# Autodesk Inventor assembly: sec_floor
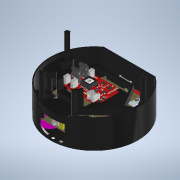
[picture p0: Inventor's stored thumbnail of the model, 180x180]
Saved by Autodesk Inventor 2020.4 (Build 244396000, 396)
## iProperties
Created: 2021-11-24
Part Number: sec_floor
Document SubType Name: Assembly
Designer: Acer
Author: Acer
## Documents named in this file (11)
- C:\Users\Acer\Documents\MATLAB\Doutorado\CAD\Inventor\sec_floor\sec_floor.iam
- C:\Users\Acer\Documents\MATLAB\Doutorado\CAD\Inventor\sec_floor\plate_sec_floor.ipt
- C:\Users\Acer\Documents\MATLAB\Doutorado\CAD\Inventor\sec_floor\SupportFirstToSecond.ipt
- C:\Users\Acer\Documents\MATLAB\Doutorado\CAD\Inventor\sec_floor\SupportSecondToCoverNew.ipt
- C:\Users\Acer\Documents\MATLAB\Doutorado\CAD\Inventor\sec_floor\MainboardSpacer.ipt
- C:\Users\Acer\Documents\MATLAB\Doutorado\CAD\Inventor\sec_floor\KickerBoard\KickerBoard_V1.1.iam
- C:\Users\Acer\Documents\MATLAB\Doutorado\CAD\Inventor\sec_floor\MainBoard\MainBoard_V1.1.iam
- C:\Users\Acer\Documents\MATLAB\Doutorado\CAD\Inventor\sec_floor\CoverNew.ipt
- C:\Users\Acer\Documents\MATLAB\Doutorado\CAD\Inventor\sec_floor\tag_green.ipt
- C:\Users\Acer\Documents\MATLAB\Doutorado\CAD\Inventor\sec_floor\tag_magenta.ipt
- C:\Users\Acer\Documents\MATLAB\Doutorado\CAD\Inventor\sec_floor\tag_yellow.ipt
## Components (19 placed, 10 different names)
1. plate_sec_floor:1 — Mate:1, Mate:2, Mate:3, Mate:4, Angle:1, Angle:2, Angle:3, Angle:4, Mate:5, Mate:6, Mate:7, Mate:8, Mate:9, Mate:10, Angle:5, Angle:6, Mate:11, Mate:12, Mate:13, Mate:14, Mate:15, Mate:16, Angle:7, Angle:8, Angle:9, Angle:10, Mate:17, Mate:18, Mate:19, Mate:20, Mate:21, Mate:22, Mate:23, Angle:11
2. SupportFirstToSecond:1 — Mate:1, Angle:4, Mate:5
3. SupportFirstToSecond:2 — Mate:2, Angle:3, Mate:8
4. SupportFirstToSecond:3 — Mate:4, Angle:1, Mate:6
5. SupportFirstToSecond:4 — Mate:3, Angle:2, Mate:7
6. SupportSecondToCoverNew:1 — Mate:9, Angle:5, Mate:12, Mate:28
7. SupportSecondToCoverNew:2 — Mate:10, Angle:6, Mate:11, Mate:27
8. MainboardSpacer:1 — Mate:13, Angle:7, Mate:19
9. MainboardSpacer:2 — Mate:14, Angle:8, Mate:17, Mate:26
10. MainboardSpacer:3 — Mate:16, Angle:9, Mate:20, Mate:24
11. MainboardSpacer:4 — Mate:15, Angle:10, Mate:18, Mate:25
12. KickerBoard_V1.1:1 [sub-assembly] — Mate:21, Mate:22, Mate:23
13. MainBoard_V1.1:1 [sub-assembly] — Mate:24, Mate:25, Mate:26
14. CoverNew:1 — Mate:27, Angle:11, Mate:28, Mate:29, Mate:30, Mate:31, Mate:32, Mate:33, Mate:34, Mate:35, Mate:36, Mate:37, Mate:38
15. tag_green:1 — Mate:31, Mate:36
16. tag_green:2 — Mate:32, Mate:35
17. tag_magenta:1 — Mate:33, Mate:37
18. tag_magenta:2 — Mate:34, Mate:38
19. tag_yellow:1 — Mate:29, Mate:30
## Relationships (49: Mate 38, Angle 11)
- Mate:1: plate_sec_floor:1 ↔ SupportFirstToSecond:1
- Mate:2: plate_sec_floor:1 ↔ SupportFirstToSecond:2
- Mate:3: plate_sec_floor:1 ↔ SupportFirstToSecond:4
- Mate:4: plate_sec_floor:1 ↔ SupportFirstToSecond:3
- Angle:1 (0 deg): plate_sec_floor:1 ↔ SupportFirstToSecond:3
- Angle:2 (0 deg): plate_sec_floor:1 ↔ SupportFirstToSecond:4
- Angle:3 (0 deg): plate_sec_floor:1 ↔ SupportFirstToSecond:2
- Angle:4 (0 deg): plate_sec_floor:1 ↔ SupportFirstToSecond:1
- Mate:5 (0.1 mm): plate_sec_floor:1 ↔ SupportFirstToSecond:1
- Mate:6: plate_sec_floor:1 ↔ SupportFirstToSecond:3
- Mate:7: plate_sec_floor:1 ↔ SupportFirstToSecond:4
- Mate:8: plate_sec_floor:1 ↔ SupportFirstToSecond:2
- Mate:9: plate_sec_floor:1 ↔ SupportSecondToCoverNew:1
- Mate:10: plate_sec_floor:1 ↔ SupportSecondToCoverNew:2
- Angle:5 (0 deg): plate_sec_floor:1 ↔ SupportSecondToCoverNew:1
- Angle:6 (0 deg): plate_sec_floor:1 ↔ SupportSecondToCoverNew:2
- Mate:11 (0.1 mm): plate_sec_floor:1 ↔ SupportSecondToCoverNew:2
- Mate:12: plate_sec_floor:1 ↔ SupportSecondToCoverNew:1
- Mate:13: plate_sec_floor:1 ↔ MainboardSpacer:1
- Mate:14: plate_sec_floor:1 ↔ MainboardSpacer:2
- Mate:15: plate_sec_floor:1 ↔ MainboardSpacer:4
- Mate:16: plate_sec_floor:1 ↔ MainboardSpacer:3
- Angle:7 (0 deg): plate_sec_floor:1 ↔ MainboardSpacer:1
- Angle:8 (0 deg): plate_sec_floor:1 ↔ MainboardSpacer:2
- Angle:9 (0 deg): plate_sec_floor:1 ↔ MainboardSpacer:3
- Angle:10 (0 deg): plate_sec_floor:1 ↔ MainboardSpacer:4
- Mate:17: plate_sec_floor:1 ↔ MainboardSpacer:2
- Mate:18: plate_sec_floor:1 ↔ MainboardSpacer:4
- Mate:19: plate_sec_floor:1 ↔ MainboardSpacer:1
- Mate:20: plate_sec_floor:1 ↔ MainboardSpacer:3
- Mate:21: plate_sec_floor:1 ↔ KickerBoard_V1.1:1
- Mate:22: plate_sec_floor:1 ↔ KickerBoard_V1.1:1
- Mate:23: plate_sec_floor:1 ↔ KickerBoard_V1.1:1
- Mate:24: MainboardSpacer:3 ↔ MainBoard_V1.1:1
- Mate:25: MainboardSpacer:4 ↔ MainBoard_V1.1:1
- Mate:26: MainboardSpacer:2 ↔ MainBoard_V1.1:1
- Mate:27: SupportSecondToCoverNew:2 ↔ CoverNew:1
- Angle:11 (0 deg): plate_sec_floor:1 ↔ CoverNew:1
- Mate:28: SupportSecondToCoverNew:1 ↔ CoverNew:1
- Mate:29: CoverNew:1 ↔ tag_yellow:1
- Mate:30: CoverNew:1 ↔ tag_yellow:1
- Mate:31: CoverNew:1 ↔ tag_green:1
- Mate:32: CoverNew:1 ↔ tag_green:2
- Mate:33: CoverNew:1 ↔ tag_magenta:1
- Mate:34: CoverNew:1 ↔ tag_magenta:2
- Mate:35: CoverNew:1 ↔ tag_green:2
- Mate:36: CoverNew:1 ↔ tag_green:1
- Mate:37: CoverNew:1 ↔ tag_magenta:1
- Mate:38: CoverNew:1 ↔ tag_magenta:2
